# Autodesk Inventor assembly: Streetlight_Sensor
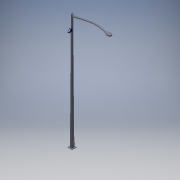
[picture p0: Inventor's stored thumbnail of the model, 180x180]
Saved by Autodesk Inventor 2019 (Build 230136000, 136)
## iProperties
Created: 2018-09-02
Part Number: Streetlight_Sensor
Document SubType Name: Assembly
Designer: Crater-Windows
Author: Crater-Windows
## Documents named in this file (5)
- C:\Users\Crater-Windows\Google Drive\Academics\William Jewell College\Extracurricular\Honors Project - DROP\DROP - Sensor Housing\Streetlight_Sensor.iam
- C:\Users\Crater-Windows\Google Drive\Academics\William Jewell College\Extracurricular\Honors Project - DROP\DROP - Sensor Housing\StreetLight.ipt
- C:\Users\Crater-Windows\Google Drive\Academics\William Jewell College\Extracurricular\Honors Project - DROP\DROP - Sensor Housing\MainHousing.ipt
- C:\Users\Crater-Windows\Google Drive\Academics\William Jewell College\Extracurricular\Honors Project - DROP\DROP - Sensor Housing\SolarPanel.ipt
- C:\Users\Crater-Windows\Google Drive\Academics\William Jewell College\Extracurricular\Honors Project - DROP\DROP - Sensor Housing\MainHousing_BottomPlate.ipt
## Components (4 placed, 4 different names)
1. StreetLight:1 — Mate:4, Angle:1, Flush:2, Flush:3
2. MainHousing:1 — Mate:1, Mate:2, Mate:3, Insert:1, Flush:1, Mate:4, Angle:1, Flush:2, Flush:3
3. SolarPanel:1 — Mate:1, Mate:2, Mate:3
4. MainHousing_BottomPlate:1 — Insert:1, Flush:1
## Relationships (9: Mate 4, Flush 3, Insert 1, Angle 1)
- Mate:1: MainHousing:1 ↔ SolarPanel:1
- Mate:2: MainHousing:1 ↔ SolarPanel:1
- Mate:3: MainHousing:1 ↔ SolarPanel:1
- Insert:1: MainHousing:1 ↔ MainHousing_BottomPlate:1
- Flush:1: MainHousing:1 ↔ MainHousing_BottomPlate:1
- Mate:4 (81.28 mm): StreetLight:1 ↔ MainHousing:1
- Angle:1 (0 deg): StreetLight:1 ↔ MainHousing:1
- Flush:2 (195.58 mm): StreetLight:1 ↔ MainHousing:1
- Flush:3 (-762 mm): StreetLight:1 ↔ MainHousing:1
